# Autodesk Inventor assembly: Flywheel w motor_MIR
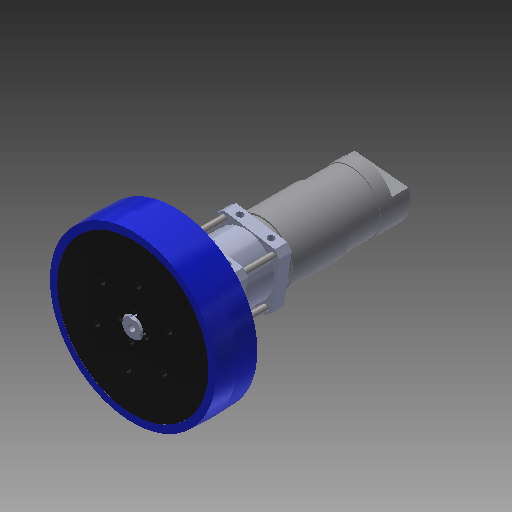
[picture p0: Inventor's stored thumbnail of the model, 512x512]
Saved by Autodesk Inventor 2017 (Build 210142000, 142)
## iProperties
Created: 2016-10-11
Part Number: Flywheel w motor_MIR
Document SubType Name: Assembly
Designer: Aditya
Author: Aditya
## Documents named in this file (4)
- C:\Users\Aditya\Documents\GitHub\RobotuxCAD\Team Robotux 15-16 Robot Cad Assets\Flywheel w motor_MIR.iam
- C:\Users\Aditya\Documents\GitHub\RobotuxCAD\Team Robotux 15-16 Robot Cad Assets\Andy Mark Parts\am-2964NeveRest-noGearbox_MIR.ipt
- C:\Users\Aditya\Documents\GitHub\RobotuxCAD\Team Robotux 15-16 Robot Cad Assets\Andy Mark Parts\am-2875+Banebots+P60+4-1_MIR.ipt
- C:\Users\Aditya\Documents\GitHub\RobotuxCAD\Team Robotux 15-16 Robot Cad Assets\Andy Mark Parts\am-2648_4inWheel8mmHubblu_MIR.ipt
## Components (3 placed, 3 different names)
1. am-2964NeveRest-noGearbox_MIR:1 — Mate:3, Mate:1
2. am-2875+Banebots+P60+4-1_MIR:1 — Mate:3, Mate:1, Mate:5, Mate:4
3. am-2648_4inWheel8mmHubblu_MIR:1 — Mate:5, Mate:4
## Relationships (4: Mate 4)
- Mate:3: am-2964NeveRest-noGearbox_MIR:1 ↔ am-2875+Banebots+P60+4-1_MIR:1
- Mate:1: am-2964NeveRest-noGearbox_MIR:1 ↔ am-2875+Banebots+P60+4-1_MIR:1
- Mate:5: am-2875+Banebots+P60+4-1_MIR:1 ↔ am-2648_4inWheel8mmHubblu_MIR:1
- Mate:4: am-2875+Banebots+P60+4-1_MIR:1 ↔ am-2648_4inWheel8mmHubblu_MIR:1
